# Autodesk Inventor assembly: BoxWIthSUpport2
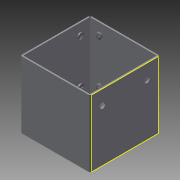
[picture p0: Inventor's stored thumbnail of the model, 180x180]
Saved by Autodesk Inventor 2013 (Build 170138000, 138)
## iProperties
Created: 2013-07-15
Part Number: BoxWIthSUpport2
Document SubType Name: Assembly
Designer: root
Author: root
## Documents named in this file (5)
- I:\FRC_Projects\Cad\Inventor_Projects\Shooter-Cleaned\HopperAssembly\TopHopper\BoxWithSupport2\BoxWIthSUpport2.iam
- I:\FRC_Projects\Cad\Inventor_Projects\Shooter-Cleaned\HopperAssembly\TopHopper\BoxWithSupport2\Box2.ipt
- I:\FRC_Projects\Cad\Inventor_Projects\Shooter-Cleaned\HopperAssembly\TopHopper\BoxWithSupport2\SideSupport.ipt
- I:\FRC_Projects\Cad\Inventor_Projects\Shooter-Cleaned\Libraries\ContentCenter\ANSI B18.6.3 - 5-44 UNF - 0.375(17).ipt
- I:\FRC_Projects\Cad\Inventor_Projects\Shooter-Cleaned\Libraries\ContentCenter\ANSI B18.6.3 - 5 - 44(2).ipt
## Components (11 placed, 4 different names)
1. Box2:1 — Mate:1, Mate:2, Mate:3, Mate:4, Mate:5, Mate:6, Mate:7, Mate:8, Mate:11, Mate:12
2. SideSupport:1 — Mate:9, Mate:10, Mate:11, Mate:19, Mate:22
3. SideSupport:2 — Mate:12, Mate:13, Mate:14, Mate:18, Mate:20
4. Cross Recessed Binding Head Machine Screw - Type II - Inch No. 5 - 44 - 3/8:1 — Mate:1, Mate:2, Mate:9, Mate:17
5. Hex Machine Screw Nut - Inch 5 - 44:1 — Mate:21, Mate:22
6. Cross Recessed Binding Head Machine Screw - Type II - Inch No. 5 - 44 - 3/8:2 — Mate:7, Mate:8, Mate:13, Mate:15
7. Cross Recessed Binding Head Machine Screw - Type II - Inch No. 5 - 44 - 3/8:4 — Mate:5, Mate:6, Mate:14, Mate:16
8. Cross Recessed Binding Head Machine Screw - Type II - Inch No. 5 - 44 - 3/8:5 — Mate:3, Mate:4, Mate:10, Mate:21
9. Hex Machine Screw Nut - Inch 5 - 44:2 — Mate:16, Mate:20
10. Hex Machine Screw Nut - Inch 5 - 44:3 — Mate:15, Mate:18
11. Hex Machine Screw Nut - Inch 5 - 44:4 — Mate:17, Mate:19
## Relationships (22: Mate 22)
- Mate:1: Box2:1 ↔ Cross Recessed Binding Head Machine Screw - Type II - Inch No. 5 - 44 - 3/8:1
- Mate:2: Box2:1 ↔ Cross Recessed Binding Head Machine Screw - Type II - Inch No. 5 - 44 - 3/8:1
- Mate:3: Box2:1 ↔ Cross Recessed Binding Head Machine Screw - Type II - Inch No. 5 - 44 - 3/8:5
- Mate:4: Box2:1 ↔ Cross Recessed Binding Head Machine Screw - Type II - Inch No. 5 - 44 - 3/8:5
- Mate:5: Box2:1 ↔ Cross Recessed Binding Head Machine Screw - Type II - Inch No. 5 - 44 - 3/8:4
- Mate:6: Box2:1 ↔ Cross Recessed Binding Head Machine Screw - Type II - Inch No. 5 - 44 - 3/8:4
- Mate:7: Box2:1 ↔ Cross Recessed Binding Head Machine Screw - Type II - Inch No. 5 - 44 - 3/8:2
- Mate:8: Box2:1 ↔ Cross Recessed Binding Head Machine Screw - Type II - Inch No. 5 - 44 - 3/8:2
- Mate:9: SideSupport:1 ↔ Cross Recessed Binding Head Machine Screw - Type II - Inch No. 5 - 44 - 3/8:1
- Mate:10: SideSupport:1 ↔ Cross Recessed Binding Head Machine Screw - Type II - Inch No. 5 - 44 - 3/8:5
- Mate:11: Box2:1 ↔ SideSupport:1
- Mate:12: Box2:1 ↔ SideSupport:2
- Mate:13: SideSupport:2 ↔ Cross Recessed Binding Head Machine Screw - Type II - Inch No. 5 - 44 - 3/8:2
- Mate:14: SideSupport:2 ↔ Cross Recessed Binding Head Machine Screw - Type II - Inch No. 5 - 44 - 3/8:4
- Mate:15: Cross Recessed Binding Head Machine Screw - Type II - Inch No. 5 - 44 - 3/8:2 ↔ Hex Machine Screw Nut - Inch 5 - 44:3
- Mate:16: Cross Recessed Binding Head Machine Screw - Type II - Inch No. 5 - 44 - 3/8:4 ↔ Hex Machine Screw Nut - Inch 5 - 44:2
- Mate:17: Cross Recessed Binding Head Machine Screw - Type II - Inch No. 5 - 44 - 3/8:1 ↔ Hex Machine Screw Nut - Inch 5 - 44:4
- Mate:18: SideSupport:2 ↔ Hex Machine Screw Nut - Inch 5 - 44:3
- Mate:19: SideSupport:1 ↔ Hex Machine Screw Nut - Inch 5 - 44:4
- Mate:20: SideSupport:2 ↔ Hex Machine Screw Nut - Inch 5 - 44:2
- Mate:21: Hex Machine Screw Nut - Inch 5 - 44:1 ↔ Cross Recessed Binding Head Machine Screw - Type II - Inch No. 5 - 44 - 3/8:5
- Mate:22: SideSupport:1 ↔ Hex Machine Screw Nut - Inch 5 - 44:1
